# Autodesk Inventor assembly: piping runs
(part 2 of 2)
Elbow45Key: v3#421a8b99-1721-409a-bc3b-c00889561754#1
_ComponentInfo: <CS><C N="Pipe" R="2.000000" IR="1.950000" PL="PL" PN="ISO 4065 Pipe 40 x 0.5 S40"><CO N="1"><FE V="0"/><FD V="0"/><ET V="Jointed"/><NS V="M40"/><MA  V="6.000000"/><MI V="1.200000"/><WP X="25.000000" Y="0.000000" Z="0.000000"/><WA X="1.000000" Y="0.000000" Z="0.000000"/></CO><CO N="2"><FE  V="0"/><FD V="1"/><ET V="Jointed"/><NS V="M40"/><MA V="6.000000"/><MI V="1.200000"/><WP X="0.000000" Y="0.000000" Z="0.000000"/><WA X="1.000000"  Y="0.000000" Z="0.000000"/></CO></C><C N="Coupling" CW="7.660000"><CO N="1"><FE V="1"/><FD V="1"/><ET V="Jointed"/><NS V="M40"/><MA V="3.830000"/><MI  V="0.766000"/><WP X="-0.000000" Y="0.000000" Z="0.000000"/><WA X="-1.000000" Y="0.000000" Z="0.000000"/></CO><CO N="2"><FE V="1"/><FD V="0"/><ET  V="Jointed"/><NS V="M40"/><MA V="3.830000"/><MI V="0.766000"/><WP X="-7.660000" Y="0.000000" Z="0.000000"/><WA X="-1.000000" Y="0.000000"  Z="0.000000"/></CO></C><C N="Elbow90" ER="3.850394" S1="7.450394" S2="7.450394" D1="3.600000" D2="3.600000"><CO N="1"><FE V="1"/><FD V="1"/><ET  V="Jointed"/><NS V="M40"/><MA V="3.600000"/><MI V="0.720000"/><WP X="7.450394" Y="0.000000" Z="7.450394"/><WA X="-1.000000" Y="0.000000"  Z="0.000000"/></CO><CO N="2"><FE V="1"/><FD V="0"/><ET V="Jointed"/><NS V="M40"/><MA V="3.600000"/><MI V="0.720000"/><WP X="-0.000000" Y="0.000000"  Z="0.000000"/><WA X="0.000000" Y="0.000000" Z="-1.000000"/></CO></C><C N="Elbow45" ER="5.674352" S1="5.950394" S2="5.950394" D1="3.600000"  D2="3.600000"><CO N="1"><FE V="1"/><FD V="1"/><ET V="Jointed"/><NS V="M40"/><MA V="3.600000"/><MI V="0.720000"/><WP X="4.207564" Y="0.000000"  Z="10.157957"/><WA X="-0.707107" Y="0.000000" Z="-0.707107"/></CO><CO N="2"><FE V="1"/><FD V="0"/><ET V="Jointed"/><NS V="M40"/><MA V="3.600000"/><MI  V="0.720000"/><WP X="-0.000000" Y="0.000000" Z="0.000000"/><WA X="0.000000" Y="0.000000" Z="-1.000000"/></CO></C></CS>
Name: Hydraulic Hose - No Fittings
_ComponentInfo: <CS><C N="Pipe" R="1.117600" OR="1.117600" IR="0.635000" PL="PL" PartType="" SymKey="" PN="Parker Hydraulic Hose - No Skive 1/2"><CO N="1"><FE V="0"/><FD V="0"/><ET V="Hose - Permanent"/><NS V="1/2"/><MA V="2.540000"/><MI V="0.508000"/><WP X="12.700000" Y="0.000000" Z="0.000000"/><WA X="1.000000" Y="0.000000" Z="0.000000"/></CO><CO N="2"><FE V="0"/><FD V="1"/><ET V="Hose - Permanent"/><NS V="1/2"/><MA V="2.540000"/><MI V="0.508000"/><WP X="0.000000" Y="0.000000" Z="0.000000"/><WA X="1.000000" Y="0.000000" Z="0.000000"/></CO></C></CS>
SuppressStartFitting: True
SuppressEndFitting: True
Author: Autodesk
## Documents named in this file (1)
- M:\AUTOBUILD\INV.Official.RTM\Application\App\Design Data\Tube & Pipe\piping runs.iam
